# Autodesk Inventor assembly: ASY TRM 020 star
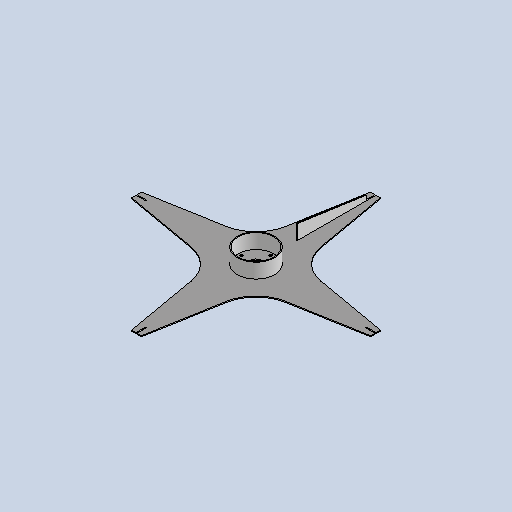
[picture p0: Inventor's stored thumbnail of the model, 512x512]
Saved by Autodesk Inventor 2025 (Build 290162010, 162A)
## iProperties
Created: 2024-09-08
Part Number: ASY TRM 020 star
Document SubType Name: Assembly
Designer: pokla
Author: pokla
## Documents named in this file (4)
- C:\Users\admin\YandexDisk-badmisterfox\домашниий пк\Inventor\BSH_Beshkino_bio_tank\ASY TRM 020 star.iam
- C:\Users\admin\YandexDisk-badmisterfox\домашниий пк\Inventor\BSH_Beshkino_bio_tank\TRM 030 star main.ipt
- C:\Users\admin\YandexDisk-badmisterfox\домашниий пк\Inventor\BSH_Beshkino_bio_tank\TRM 032 contrforce ring.ipt
- C:\Users\admin\YandexDisk-badmisterfox\домашниий пк\Inventor\BSH_Beshkino_bio_tank\TRM 030 star conrtforce plate.ipt
## Components (3 placed, 3 different names)
1. TRM 030 star main:1
2. TRM 032 contrforce ring:1
3. TRM 030 star conrtforce plate:1
## Relationships (2: RevoluteJoint 1, WeldJoint 1)
- [RevoluteJoint]: TRM 030 star main:1 ↔ TRM 032 contrforce ring:1
- [WeldJoint]: TRM 030 star main:1 ↔ TRM 030 star conrtforce plate:1
